# Autodesk Inventor assembly: Ensamble Mecanismo cilindro
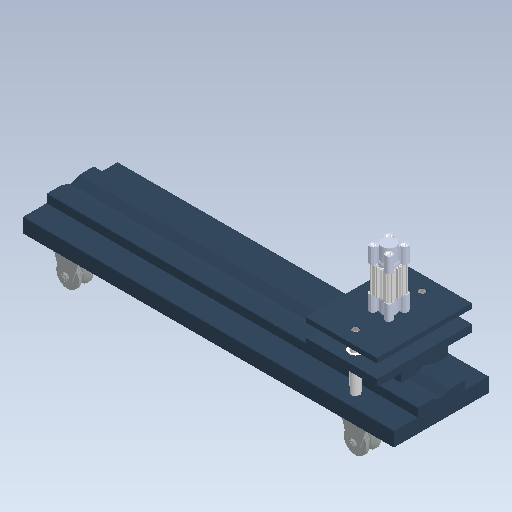
[picture p0: Inventor's stored thumbnail of the model, 512x512]
Saved by Autodesk Inventor 2021 (Build 250183000, 183)
## iProperties
Created: 2020-01-15
Part Number: Ensamble Mecanismo cilindro
Document SubType Name: Assembly
Designer: Nelson
Mass: 184587 g
Surface Area: 10520.7 cm^2
Volume: 24885.7 cm^3
Density: 7.41741 g/cm^3
Sending System: SolidWorks 2020
Last Author: Micro
Last Saved: 2020-01-16
Author: Nelson
## Documents named in this file (12)
- D:\Nelson\Documentos\Inventor\PrensaHidraulica_Automatizada\Ensamble Mecanismo cilindro.iam
- Ensamble mecanismo cilindro.iam
- D:\Nelson\Documentos\Inventor\PrensaHidraulica_Automatizada\Base soporte tubos.ipt
- D:\Nelson\Documentos\Inventor\PrensaHidraulica_Automatizada\Eje roscado base soporte tubo.ipt
- D:\Nelson\Documentos\Inventor\PrensaHidraulica_Automatizada\Soporte Piston.ipt
- D:\Nelson\Documentos\Inventor\PrensaHidraulica_Automatizada\Soporte Superior Tubos.ipt
- D:\Nelson\Documentos\Inventor\PrensaHidraulica_Automatizada\Buje soporte superior.ipt
- D:\Nelson\Documentos\Inventor\PrensaHidraulica_Automatizada\DIN 7984 - M8 x 20.ipt
- D:\Nelson\Documentos\Inventor\PrensaHidraulica_Automatizada\V-Groove_Roller.ipt
- D:\Nelson\Documentos\Inventor\Content Center Files\R2021\en-US\DIN 933\DIN 933 - M6  x 12.ipt
- D:\Nelson\Documentos\Inventor\PrensaHidraulica_Automatizada\04766013.iam
- D:\Nelson\Documentos\Inventor\PrensaHidraulica_Automatizada\DIN EN ISO 4762 - M6 x 50.ipt
## Components (36 placed, 10 different names)
1. Base soporte tubos:1 — Mate:27, Mate:28, Mate:30, Mate:47, Mate:61, Mate:62, Mate:63, Mate:64, Mate:65, Mate:66, Mate:67, Mate:68, Mate:69, Mate:70, Mate:71, Mate:72
2. Eje roscado base soporte tubo:1 — Mate:27, Mate:28, Mate:48, Mate:56, Mate:57
3. Eje roscado base soporte tubo:2 — Mate:30, Mate:47, Mate:49, Mate:58
4. Soporte Piston:1 — Mate:56, Mate:57, Mate:58, Mate:59, Mate:60, Flush:1, Flush:2, Mate:106, Mate:108, Mate:109, Mate:110, Mate:113, Mate:114, Mate:115, Mate:116, Mate:117, Mate:118, Mate:119, Mate:120
5. Soporte Superior Tubos:1 — Mate:36, Mate:37, Mate:38, Mate:39, Mate:40, Mate:41, Mate:42, Mate:43, Mate:111, Mate:112
6. Buje soporte superior:1 — Mate:38, Mate:39, Mate:49
7. Buje soporte superior:2 — Mate:36, Mate:37, Mate:48
8. Buje soporte superior:3 — Mate:40, Mate:41
9. Buje soporte superior:4 — Mate:42, Mate:43
10. DIN 7984 M8 x 20:1 — Mate:59, Flush:1
11. DIN 7984 M8 x 20:2 — Mate:60, Flush:2
12. V-Groove_Roller:1 — Mate:62, Mate:65, Mate:66, Mate:93, Mate:94, Mate:95, Mate:96, Mate:102, Mate:103, Mate:104, Mate:105
13. V-Groove_Roller:2 — Mate:61, Mate:69, Mate:70, Mate:89, Mate:90, Mate:91, Mate:92, Mate:97, Mate:99, Mate:100, Mate:101
14. V-Groove_Roller:3 — Mate:63, Mate:67, Mate:68, Mate:81, Mate:82, Mate:83, Mate:84, Mate:85, Mate:86, Mate:87, Mate:88
15. V-Groove_Roller:4 — Mate:64, Mate:71, Mate:72, Mate:73, Mate:74, Mate:75, Mate:76, Mate:77, Mate:78, Mate:79, Mate:80
16. DIN 933 - replaced by DIN EN 24017 M6  x 12:1 — Mate:73, Mate:74
17. DIN 933 - replaced by DIN EN 24017 M6  x 12:2 — Mate:76, Mate:80
18. DIN 933 - replaced by DIN EN 24017 M6  x 12:3 — Mate:75, Mate:79
19. DIN 933 - replaced by DIN EN 24017 M6  x 12:4 — Mate:77, Mate:78
20. DIN 933 - replaced by DIN EN 24017 M6  x 12:5 — Mate:81, Mate:82
21. DIN 933 - replaced by DIN EN 24017 M6  x 12:6 — Mate:87, Mate:88
22. DIN 933 - replaced by DIN EN 24017 M6  x 12:7 — Mate:83, Mate:84
23. DIN 933 - replaced by DIN EN 24017 M6  x 12:8 — Mate:85, Mate:86
24. DIN 933 - replaced by DIN EN 24017 M6  x 12:9 — Mate:89, Mate:101
25. DIN 933 - replaced by DIN EN 24017 M6  x 12:10 — Mate:92, Mate:99
26. DIN 933 - replaced by DIN EN 24017 M6  x 12:11 — Mate:90, Mate:100
27. DIN 933 - replaced by DIN EN 24017 M6  x 12:12 — Mate:91, Mate:97
28. DIN 933 - replaced by DIN EN 24017 M6  x 12:13 — Mate:93, Mate:105
29. DIN 933 - replaced by DIN EN 24017 M6  x 12:14 — Mate:96, Mate:102
30. DIN 933 - replaced by DIN EN 24017 M6  x 12:15 — Mate:94, Mate:104
31. DIN 933 - replaced by DIN EN 24017 M6  x 12:16 — Mate:95, Mate:103
32. 04766013:2 [sub-assembly] — Mate:106, Mate:108, Mate:109, Mate:110, Mate:111, Mate:112
33. DIN EN ISO 4762 M6 x 50:1 — Mate:113, Mate:120
34. DIN EN ISO 4762 M6 x 50:2 — Mate:114, Mate:117
35. DIN EN ISO 4762 M6 x 50:3 — Mate:115, Mate:119
36. DIN EN ISO 4762 M6 x 50:4 — Mate:116, Mate:118
## Relationships (79: Mate 77, Flush 2)
- Mate:27: Base soporte tubos:1 ↔ Eje roscado base soporte tubo:1
- Mate:28: Base soporte tubos:1 ↔ Eje roscado base soporte tubo:1
- Mate:30: Base soporte tubos:1 ↔ Eje roscado base soporte tubo:2
- Mate:36: Soporte Superior Tubos:1 ↔ Buje soporte superior:2
- Mate:37: Soporte Superior Tubos:1 ↔ Buje soporte superior:2
- Mate:38: Soporte Superior Tubos:1 ↔ Buje soporte superior:1
- Mate:39: Soporte Superior Tubos:1 ↔ Buje soporte superior:1
- Mate:40: Soporte Superior Tubos:1 ↔ Buje soporte superior:3
- Mate:41: Soporte Superior Tubos:1 ↔ Buje soporte superior:3
- Mate:42: Soporte Superior Tubos:1 ↔ Buje soporte superior:4
- Mate:43: Soporte Superior Tubos:1 ↔ Buje soporte superior:4
- Mate:47: Base soporte tubos:1 ↔ Eje roscado base soporte tubo:2
- Mate:48: Eje roscado base soporte tubo:1 ↔ Buje soporte superior:2
- Mate:49: Eje roscado base soporte tubo:2 ↔ Buje soporte superior:1
- Mate:56: Eje roscado base soporte tubo:1 ↔ Soporte Piston:1
- Mate:57: Eje roscado base soporte tubo:1 ↔ Soporte Piston:1
- Mate:58: Eje roscado base soporte tubo:2 ↔ Soporte Piston:1
- Mate:59: Soporte Piston:1 ↔ DIN 7984 M8 x 20:1
- Mate:60: Soporte Piston:1 ↔ DIN 7984 M8 x 20:2
- Flush:1: Soporte Piston:1 ↔ DIN 7984 M8 x 20:1
- Flush:2: Soporte Piston:1 ↔ DIN 7984 M8 x 20:2
- Mate:61: Base soporte tubos:1 ↔ V-Groove_Roller:2
- Mate:62: Base soporte tubos:1 ↔ V-Groove_Roller:1
- Mate:63: Base soporte tubos:1 ↔ V-Groove_Roller:3
- Mate:64: Base soporte tubos:1 ↔ V-Groove_Roller:4
- Mate:65: Base soporte tubos:1 ↔ V-Groove_Roller:1
- Mate:66: Base soporte tubos:1 ↔ V-Groove_Roller:1
- Mate:67: Base soporte tubos:1 ↔ V-Groove_Roller:3
- Mate:68: Base soporte tubos:1 ↔ V-Groove_Roller:3
- Mate:69: Base soporte tubos:1 ↔ V-Groove_Roller:2
- Mate:70: Base soporte tubos:1 ↔ V-Groove_Roller:2
- Mate:71: Base soporte tubos:1 ↔ V-Groove_Roller:4
- Mate:72: Base soporte tubos:1 ↔ V-Groove_Roller:4
- Mate:73: V-Groove_Roller:4 ↔ DIN 933 - replaced by DIN EN 24017 M6  x 12:1
- Mate:74: V-Groove_Roller:4 ↔ DIN 933 - replaced by DIN EN 24017 M6  x 12:1
- Mate:75: V-Groove_Roller:4 ↔ DIN 933 - replaced by DIN EN 24017 M6  x 12:3
- Mate:76: V-Groove_Roller:4 ↔ DIN 933 - replaced by DIN EN 24017 M6  x 12:2
- Mate:77: V-Groove_Roller:4 ↔ DIN 933 - replaced by DIN EN 24017 M6  x 12:4
- Mate:78: V-Groove_Roller:4 ↔ DIN 933 - replaced by DIN EN 24017 M6  x 12:4
- Mate:79: V-Groove_Roller:4 ↔ DIN 933 - replaced by DIN EN 24017 M6  x 12:3
- Mate:80: V-Groove_Roller:4 ↔ DIN 933 - replaced by DIN EN 24017 M6  x 12:2
- Mate:81: V-Groove_Roller:3 ↔ DIN 933 - replaced by DIN EN 24017 M6  x 12:5
- Mate:82: V-Groove_Roller:3 ↔ DIN 933 - replaced by DIN EN 24017 M6  x 12:5
- Mate:83: V-Groove_Roller:3 ↔ DIN 933 - replaced by DIN EN 24017 M6  x 12:7
- Mate:84: V-Groove_Roller:3 ↔ DIN 933 - replaced by DIN EN 24017 M6  x 12:7
- Mate:85: V-Groove_Roller:3 ↔ DIN 933 - replaced by DIN EN 24017 M6  x 12:8
- Mate:86: V-Groove_Roller:3 ↔ DIN 933 - replaced by DIN EN 24017 M6  x 12:8
- Mate:87: V-Groove_Roller:3 ↔ DIN 933 - replaced by DIN EN 24017 M6  x 12:6
- Mate:88: V-Groove_Roller:3 ↔ DIN 933 - replaced by DIN EN 24017 M6  x 12:6
- Mate:89: V-Groove_Roller:2 ↔ DIN 933 - replaced by DIN EN 24017 M6  x 12:9
- Mate:90: V-Groove_Roller:2 ↔ DIN 933 - replaced by DIN EN 24017 M6  x 12:11
- Mate:91: V-Groove_Roller:2 ↔ DIN 933 - replaced by DIN EN 24017 M6  x 12:12
- Mate:92: V-Groove_Roller:2 ↔ DIN 933 - replaced by DIN EN 24017 M6  x 12:10
- Mate:93: V-Groove_Roller:1 ↔ DIN 933 - replaced by DIN EN 24017 M6  x 12:13
- Mate:94: V-Groove_Roller:1 ↔ DIN 933 - replaced by DIN EN 24017 M6  x 12:15
- Mate:95: V-Groove_Roller:1 ↔ DIN 933 - replaced by DIN EN 24017 M6  x 12:16
- Mate:96: V-Groove_Roller:1 ↔ DIN 933 - replaced by DIN EN 24017 M6  x 12:14
- Mate:97: V-Groove_Roller:2 ↔ DIN 933 - replaced by DIN EN 24017 M6  x 12:12
- Mate:99: V-Groove_Roller:2 ↔ DIN 933 - replaced by DIN EN 24017 M6  x 12:10
- Mate:100: V-Groove_Roller:2 ↔ DIN 933 - replaced by DIN EN 24017 M6  x 12:11
- Mate:101: V-Groove_Roller:2 ↔ DIN 933 - replaced by DIN EN 24017 M6  x 12:9
- Mate:102: V-Groove_Roller:1 ↔ DIN 933 - replaced by DIN EN 24017 M6  x 12:14
- Mate:103: V-Groove_Roller:1 ↔ DIN 933 - replaced by DIN EN 24017 M6  x 12:16
- Mate:104: V-Groove_Roller:1 ↔ DIN 933 - replaced by DIN EN 24017 M6  x 12:15
- Mate:105: V-Groove_Roller:1 ↔ DIN 933 - replaced by DIN EN 24017 M6  x 12:13
- Mate:106: Soporte Piston:1 ↔ 04766013:2
- Mate:108: Soporte Piston:1 ↔ 04766013:2
- Mate:109: Soporte Piston:1 ↔ 04766013:2
- Mate:110: Soporte Piston:1 ↔ 04766013:2
- Mate:111: Soporte Superior Tubos:1 ↔ 04766013:2
- Mate:112 (-10 mm): Soporte Superior Tubos:1 ↔ 04766013:2
- Mate:113: Soporte Piston:1 ↔ DIN EN ISO 4762 M6 x 50:1
- Mate:114: Soporte Piston:1 ↔ DIN EN ISO 4762 M6 x 50:2
- Mate:115: Soporte Piston:1 ↔ DIN EN ISO 4762 M6 x 50:3
- Mate:116: Soporte Piston:1 ↔ DIN EN ISO 4762 M6 x 50:4
- Mate:117: Soporte Piston:1 ↔ DIN EN ISO 4762 M6 x 50:2
- Mate:118: Soporte Piston:1 ↔ DIN EN ISO 4762 M6 x 50:4
- Mate:119: Soporte Piston:1 ↔ DIN EN ISO 4762 M6 x 50:3
- Mate:120: Soporte Piston:1 ↔ DIN EN ISO 4762 M6 x 50:1
